# Autodesk Inventor assembly: sideFacing
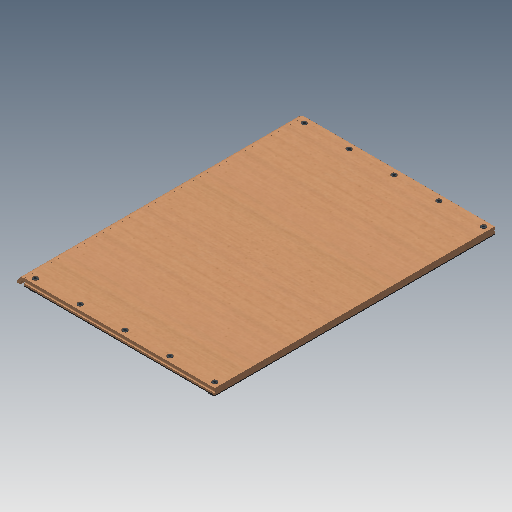
[picture p0: Inventor's stored thumbnail of the model, 512x512]
Saved by Autodesk Inventor 2018.2 (Build 222227000, 227)
## iProperties
Created: 2016-04-01
Part Number: sideFacing
Document SubType Name: Assembly
Designer: sawai
Author: sawai
## Documents named in this file (7)
- C:\Users\sawaiz\OneDrive\projects\modularRICHFrame\facing\sideFacing.iam
- C:\Users\sawaiz\OneDrive\projects\modularRICHFrame\facing\sideFace.ipt
- C:\Users\sawaiz\OneDrive\projects\modularRICHFrame\facing\sideGasket.ipt
- C:\Users\sawaiz\OneDrive\projects\modularRICHFrame\facing\sideMoulding.ipt
- C:\Users\sawaiz\OneDrive\projects\modularRICHFrame\hardware\m5TNut.ipt
- C:\Users\sawaiz\OneDrive\projects\modularRICHFrame\hardware\m5x12BlackSocketHead.ipt
- C:\Users\sawaiz\OneDrive\projects\modularRICHFrame\modularRICHFrame.xlsx
## Components (23 placed, 5 different names)
1. sideFace:1 — Mate:1, Mate:2, Mate:3, Mate:4, Flush:2, Mate:5, Flush:3, Angle:1, Angle:2, Angle:3
2. sideGasket:1 — Mate:1, Mate:2, Mate:3, Flush:1, Mate:7
3. sideMoulding:1 — Mate:4, Flush:1, Flush:2
4. m5x12BlackSocketHead:1 — Mate:5, Flush:3, Mate:6
5. m5x12BlackSocketHead:2
6. m5x12BlackSocketHead:3 — Mate:8
7. m5x12BlackSocketHead:4
8. m5x12BlackSocketHead:5
9. m5x12BlackSocketHead:6
10. m5x12BlackSocketHead:7
11. m5x12BlackSocketHead:8
12. m5x12BlackSocketHead:9
13. m5x12BlackSocketHead:10
14. m5TNut:1 — Mate:6, Angle:1, Mate:7, Angle:2, Flush:4
15. m5TNut:2
16. m5TNut:3
17. m5TNut:4
18. m5TNut:5 — Mate:8, Angle:3, Flush:4
19. m5TNut:6
20. m5TNut:7
21. m5TNut:8
22. m5TNut:9
23. m5TNut:10
## Component patterns: (10 elements, first: m5x12BlackSocketHead:1), (4 elements, first: m5TNut:1), (6 elements, first: m5TNut:5)
## Relationships (15: Mate 8, Flush 4, Angle 3)
- Mate:1: sideFace:1 ↔ sideGasket:1
- Mate:2: sideFace:1 ↔ sideGasket:1
- Mate:3: sideFace:1 ↔ sideGasket:1
- Mate:4: sideFace:1 ↔ sideMoulding:1
- Flush:1: sideGasket:1 ↔ sideMoulding:1
- Flush:2: sideFace:1 ↔ sideMoulding:1
- Mate:5: sideFace:1 ↔ m5x12BlackSocketHead:1
- Flush:3: sideFace:1 ↔ m5x12BlackSocketHead:1
- Mate:6: m5x12BlackSocketHead:1 ↔ m5TNut:1
- Angle:1 (0 deg): sideFace:1 ↔ m5TNut:1
- Mate:7 (2 mm): sideGasket:1 ↔ m5TNut:1
- Angle:2 (0 deg): sideFace:1 ↔ m5TNut:1
- Mate:8: m5x12BlackSocketHead:3 ↔ m5TNut:5
- Angle:3 (0 deg): sideFace:1 ↔ m5TNut:5
- Flush:4: m5TNut:1 ↔ m5TNut:5
## Named parameters: width = 300 mm, height = 300 mm, depth = 500 mm, facingThickness = 12.7 mm, facingGasketThickness = 1.5875 mm
